# Autodesk Inventor assembly: Handle_2_Asm
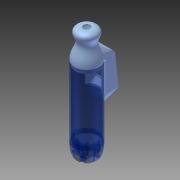
[picture p0: Inventor's stored thumbnail of the model, 180x180]
Saved by Autodesk Inventor 2011 SP2 (Build 150309200, 309)
## iProperties
Created: 2012-03-18
Part Number: Handle_2_Asm
Document SubType Name: Assembly
Designer: sungwook
Author: sungwook
## Documents named in this file (5)
- C:\Users\sungwook\Documents\Inventor\Micron20\Parts\Handle\Ver2(Al_RP)\Handle_2_Asm.iam
- C:\Users\sungwook\Documents\Inventor\Micron20\Parts\Handle\Ver2(Al_RP)\Main_Tubing_Al.ipt
- C:\Users\sungwook\Documents\Inventor\Micron20\Parts\Handle\Ver2(Al_RP)\Handle_2_Rev_Front.ipt
- C:\Users\sungwook\Documents\Inventor\Micron20\Parts\Handle\Ver2(Al_RP)\Handle_2_Back_Upper.ipt
- C:\Users\sungwook\Documents\Inventor\Micron20\Parts\Handle\Ver2(Al_RP)\Handle_2_Back_Bottom.ipt
## Components (4 placed, 4 different names)
1. Main_Tubing_Al:1 — Flush:1, Mate:1, Mate:2, Flush:2, Flush:3, Mate:7, Mate:8
2. Handle_2_Rev_Front:1 — Flush:1, Mate:1, Mate:2
3. Handle_2_Back_Upper:1 — Flush:2, Mate:3, Mate:4, Mate:5, Mate:6, Mate:7, Mate:8
4. Handle_2_Back_Bottom:1 — Flush:3, Mate:3, Mate:4, Mate:5, Mate:6
## Relationships (11: Mate 8, Flush 3)
- Flush:1: Main_Tubing_Al:1 ↔ Handle_2_Rev_Front:1
- Mate:1: Main_Tubing_Al:1 ↔ Handle_2_Rev_Front:1
- Mate:2: Main_Tubing_Al:1 ↔ Handle_2_Rev_Front:1
- Flush:2: Main_Tubing_Al:1 ↔ Handle_2_Back_Upper:1
- Flush:3: Main_Tubing_Al:1 ↔ Handle_2_Back_Bottom:1
- Mate:3: Handle_2_Back_Upper:1 ↔ Handle_2_Back_Bottom:1
- Mate:4: Handle_2_Back_Upper:1 ↔ Handle_2_Back_Bottom:1
- Mate:5: Handle_2_Back_Upper:1 ↔ Handle_2_Back_Bottom:1
- Mate:6: Handle_2_Back_Upper:1 ↔ Handle_2_Back_Bottom:1
- Mate:7: Main_Tubing_Al:1 ↔ Handle_2_Back_Upper:1
- Mate:8: Main_Tubing_Al:1 ↔ Handle_2_Back_Upper:1
